# Autodesk Inventor assembly: leg_2
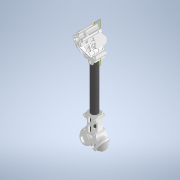
[picture p0: Inventor's stored thumbnail of the model, 180x180]
Saved by Autodesk Inventor 2020 (Build 240168000, 168)
## iProperties
Created: 2020-09-02
Part Number: leg_2
Document SubType Name: Assembly
Designer: psrobotics
Author: psrobotics
## Documents named in this file (6)
- D:\projects-3\biped_gen1\sim\model\leg_2dof_urdf\leg_2.iam
- D:\projects-3\biped_gen1\hardware\joint_connector_4_lit.ipt
- D:\projects-3\biped_gen1\hardware\joint_connector_5_lit.ipt
- D:\projects-3\biped_gen1\hardware\carbon_fiber_25_21_300.ipt
- D:\projects-3\biped_gen1\hardware\joint_connector_6.ipt
- D:\projects-3\biped_gen1\hardware\foot_ass.iam
## Components (5 placed, 5 different names)
1. joint_connector_4_lit:1 — Insert:1, Insert:2, Insert:3, Insert:4, Insert:5
2. joint_connector_5_lit:1 — Insert:1, Insert:2
3. carbon_fiber_25_21_300:1 — Insert:3, Insert:6
4. joint_connector_6:1 — Insert:4, Insert:5, Flush:1
5. foot_ass:1 [sub-assembly] — Insert:6, Flush:1
## Relationships (7: Insert 6, Flush 1)
- Insert:1: joint_connector_4_lit:1 ↔ joint_connector_5_lit:1
- Insert:2: joint_connector_4_lit:1 ↔ joint_connector_5_lit:1
- Insert:3: joint_connector_4_lit:1 ↔ carbon_fiber_25_21_300:1
- Insert:4: joint_connector_4_lit:1 ↔ joint_connector_6:1
- Insert:5: joint_connector_4_lit:1 ↔ joint_connector_6:1
- Insert:6: carbon_fiber_25_21_300:1 ↔ foot_ass:1
- Flush:1: joint_connector_6:1 ↔ foot_ass:1
